# Autodesk Inventor assembly: Toolhead_PCB
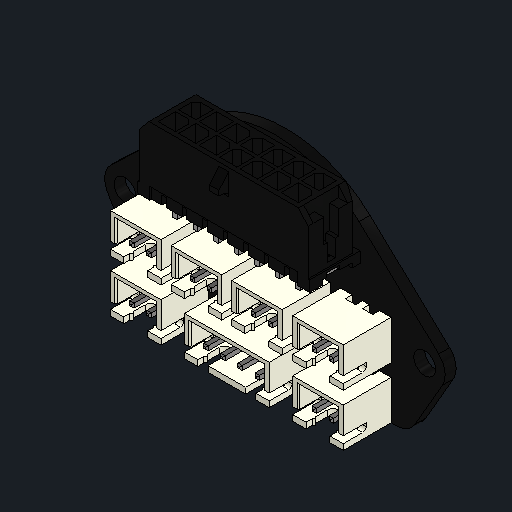
[picture p0: Inventor's stored thumbnail of the model, 512x512]
Saved by Autodesk Inventor 2025.1 (Build 291241020, 241B)
## iProperties
Company: A Company
Created: 2021-06-02
Part Number: Toolhead_PCB
Description: KiCad electronic assembly
Document SubType Name: Assembly
Designer: Joshua Eah
Authority: Unknown
Sending System: KiCad to STEP converter
Preprocessor: Open CASCADE STEP processor 6.9
Title: Toolhead_PCB.step
Author: An Author
## Documents named in this file (5)
- C:\Users\Joshua Eah\Documents\Voron 0.2\CAD\Master Assembly\Toolhead\Parts\Toolhead_PCB.iam
- C:\Users\Joshua Eah\Documents\Voron 0.2\CAD\Master Assembly\Toolhead\Parts\Umbilical Toolhead PCB\COMPOUND.ipt
- C:\Users\Joshua Eah\Documents\Voron 0.2\CAD\Master Assembly\Toolhead\Parts\Umbilical Toolhead PCB\SOLID_2.ipt
- C:\Users\Joshua Eah\Documents\Voron 0.2\CAD\Master Assembly\Toolhead\Parts\Umbilical Toolhead PCB\SOLID.ipt
- C:\Users\Joshua Eah\Documents\Voron 0.2\CAD\Master Assembly\Toolhead\Parts\Umbilical Toolhead PCB\SOLID_1.ipt
## Components (9 placed, 9 different names)
1. 2
2. 3
3. 4
4. 6
5. 7
6. 8
7. 9
8. 11
9. 12
## Named parameters: Finish3_Area = 23.7764
note: some values were not read from the file. Shown as the stored number, unit unknown: "Finish3_Area".
